# Autodesk Inventor assembly: DannyLift
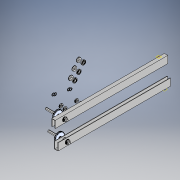
[picture p0: Inventor's stored thumbnail of the model, 180x180]
Saved by Autodesk Inventor 2018 (Build 220112000, 112)
## iProperties
Created: 2019-01-13
Part Number: DannyLift
Document SubType Name: Assembly
Designer: Gabriel
Author: Gabriel
## Documents named in this file (7)
- C:\Users\Gabriel\Documents\DannyLift.iam
- C:\Users\Gabriel\Documents\36in Aluminum Channel.ipt
- C:\Users\Gabriel\Documents\50t_20dp_gear.ipt
- C:\Users\Gabriel\Documents\half_inch_collar.ipt
- C:\Users\Gabriel\Documents\spacer.ipt
- C:\Users\Gabriel\Documents\Sanded Hex Rod.ipt
- C:\Users\Gabriel\Documents\0_500_ID_x_1_125_OD_x_0_313_WD_Flanged_Bearing_217-2731.ipt
## Components (28 placed, 6 different names)
1. 36in Aluminum Channel:1 — Mate:1, Mate:2, Mate:3, Mate:4
2. 50t_20dp_gear:1 — Mate:10, Mate:11
3. half_inch_collar:1
4. spacer:1 — Mate:12, Mate:13
5. 36in Aluminum Channel:2 — Mate:5, Mate:6, Mate:7, Mate:8
6. 50t_20dp_gear:2 — Mate:14, Mate:15
7. half_inch_collar:2
8. spacer:2 — Mate:9
9. half_inch_collar:3
10. spacer:3
11. half_inch_collar:4
12. spacer:4
13. half_inch_collar:5
14. spacer:5
15. half_inch_collar:6
16. spacer:6
17. Sanded Hex Rod:1 — Mate:9, Mate:10, Mate:11
18. Sanded Hex Rod:2 — Mate:12, Mate:13, Mate:14, Mate:15
19. 0_500_ID_x_1_125_OD_x_0_313_WD_Flanged_Bearing_217-2731:1 — Mate:5, Mate:6
20. 0_500_ID_x_1_125_OD_x_0_313_WD_Flanged_Bearing_217-2731:2 — Mate:1, Mate:2
21. 0_500_ID_x_1_125_OD_x_0_313_WD_Flanged_Bearing_217-2731:3 — Mate:7, Mate:8
22. 0_500_ID_x_1_125_OD_x_0_313_WD_Flanged_Bearing_217-2731:4 — Mate:3, Mate:4
23. 0_500_ID_x_1_125_OD_x_0_313_WD_Flanged_Bearing_217-2731:5
24. 0_500_ID_x_1_125_OD_x_0_313_WD_Flanged_Bearing_217-2731:6
25. 0_500_ID_x_1_125_OD_x_0_313_WD_Flanged_Bearing_217-2731:7
26. 0_500_ID_x_1_125_OD_x_0_313_WD_Flanged_Bearing_217-2731:8
27. 0_500_ID_x_1_125_OD_x_0_313_WD_Flanged_Bearing_217-2731:9
28. 0_500_ID_x_1_125_OD_x_0_313_WD_Flanged_Bearing_217-2731:10
## Relationships (15: Mate 15)
- Mate:1: 36in Aluminum Channel:1 ↔ 0_500_ID_x_1_125_OD_x_0_313_WD_Flanged_Bearing_217-2731:2
- Mate:2: 36in Aluminum Channel:1 ↔ 0_500_ID_x_1_125_OD_x_0_313_WD_Flanged_Bearing_217-2731:2
- Mate:3: 36in Aluminum Channel:1 ↔ 0_500_ID_x_1_125_OD_x_0_313_WD_Flanged_Bearing_217-2731:4
- Mate:4: 36in Aluminum Channel:1 ↔ 0_500_ID_x_1_125_OD_x_0_313_WD_Flanged_Bearing_217-2731:4
- Mate:5: 36in Aluminum Channel:2 ↔ 0_500_ID_x_1_125_OD_x_0_313_WD_Flanged_Bearing_217-2731:1
- Mate:6: 36in Aluminum Channel:2 ↔ 0_500_ID_x_1_125_OD_x_0_313_WD_Flanged_Bearing_217-2731:1
- Mate:7: 36in Aluminum Channel:2 ↔ 0_500_ID_x_1_125_OD_x_0_313_WD_Flanged_Bearing_217-2731:3
- Mate:8: 36in Aluminum Channel:2 ↔ 0_500_ID_x_1_125_OD_x_0_313_WD_Flanged_Bearing_217-2731:3
- Mate:9: spacer:2 ↔ Sanded Hex Rod:1
- Mate:10: 50t_20dp_gear:1 ↔ Sanded Hex Rod:1
- Mate:11: 50t_20dp_gear:1 ↔ Sanded Hex Rod:1
- Mate:12: spacer:1 ↔ Sanded Hex Rod:2
- Mate:13: spacer:1 ↔ Sanded Hex Rod:2
- Mate:14: 50t_20dp_gear:2 ↔ Sanded Hex Rod:2
- Mate:15: 50t_20dp_gear:2 ↔ Sanded Hex Rod:2
